# Autodesk Inventor assembly: pg71 and 9015 motor and 1-2 hex output shaft
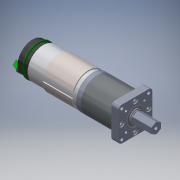
[picture p0: Inventor's stored thumbnail of the model, 180x180]
Saved by Autodesk Inventor 2018 (Build 220112000, 112)
## iProperties
Created: 2020-01-31
Part Number: pg71 and 9015 motor and 1-2 hex output shaft
Document SubType Name: Assembly
Designer: s-2513225
Author: s-2513225
## Documents named in this file (3)
- \\studenthome\students\S-2513225\GitHub\2020CAD\Over bumper intake\Parts\pg71 and 9015 motor and 1-2 hex output shaft.iam
- H:\GitHub\2020CAD\Over bumper intake\Parts\pg71 and 9015 motor and 1-2 hex output shaft.iam
- \\studenthome\students\S-2513225\GitHub\2020CAD\Over bumper intake\Parts\am-3655 PG71 500 hex Motor Encoder.ipt
## Components (2 placed, 2 different names)
1. am-3655 PG71 500 hex Motor Encoder:1
2. pg71 and 9015 motor and 1-2 hex output shaft:1 [sub-assembly]
## Relationships (2: Mate 2)
- [Mate]: am-3655 PG71 500 hex Motor Encoder:1 ↔ pg71 and 9015 motor and 1-2 hex output shaft:1
- [Mate]: am-3655 PG71 500 hex Motor Encoder:1 ↔ pg71 and 9015 motor and 1-2 hex output shaft:1
